# Autodesk Inventor assembly: Assembly1
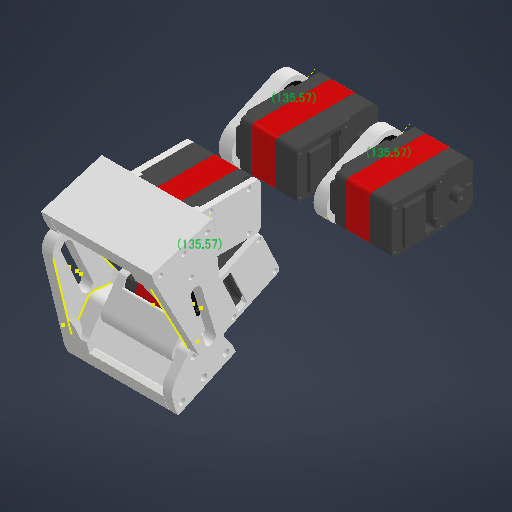
[picture p0: Inventor's stored thumbnail of the model, 512x512]
Saved by Autodesk Inventor 2026 (Build 300175000, 175)
## iProperties
Created: 2025-12-05
Part Number: Assembly1
Document SubType Name: Assembly
Designer: numai
Author: numai
## Documents named in this file (8)
- C:\Users\numai\Documents\workspace\inventor\feetech_slider_3dprint\Assembly1.iam
- C:\Users\numai\Documents\workspace\inventor\feetech_slider_3dprint\HLS3950M.ipt
- C:\Users\numai\Documents\workspace\inventor\feetech_slider_3dprint\ARRMA_1_7_25t_servo_arm.ipt
- C:\Users\numai\Documents\workspace\inventor\feetech_slider_3dprint\servo_side_plate1.ipt
- C:\Users\numai\Documents\workspace\inventor\feetech_slider_3dprint\servo_side_plate2.ipt
- C:\Users\numai\Documents\workspace\inventor\feetech_slider_3dprint\guideline.ipt
- C:\Users\numai\Documents\workspace\inventor\feetech_slider_3dprint\guideline_mir.ipt
- C:\Users\numai\Documents\workspace\inventor\feetech_slider_3dprint\arrma_boolean.ipt
## Components (17 placed, 7 different names)
1. HLS3950M:1 — メイト:1, メイト:2, フラッシュ:1, フラッシュ:2, フラッシュ:3, メイト:9, フラッシュ:4, フラッシュ:5
2. ARRMA_1_7_25t_servo_arm:1 — メイト:1, メイト:2, メイト:4
3. servo_side_plate1:1 — フラッシュ:1, フラッシュ:2
4. servo_side_plate2:1 — フラッシュ:3, メイト:23
5. guideline:1 — メイト:4, メイト:6, メイト:7, メイト:8
6. guideline_mir:1 — メイト:6, メイト:7, メイト:8, メイト:23
7. HLS3950M:2 — メイト:9, フラッシュ:4, フラッシュ:5, フラッシュ:6, フラッシュ:7, メイト:10, メイト:11, メイト:21, フラッシュ:8
8. HLS3950M:3 — フラッシュ:6, フラッシュ:7, メイト:12, メイト:13
9. ARRMA_1_7_25t_servo_arm:2 — メイト:10, メイト:11, メイト:14, メイト:18, メイト:19, メイト:20
10. ARRMA_1_7_25t_servo_arm:3 — メイト:12, メイト:13, メイト:14, メイト:15, メイト:16, メイト:17
11. arrma_boolean:1 — メイト:15, メイト:16, メイト:17, メイト:21
12. arrma_boolean:2 — メイト:18, メイト:19, メイト:20, メイト:24, フラッシュ:25
13. HLS3950M:4 — フラッシュ:8, メイト:24, フラッシュ:25, メイト:25, メイト:26, 角度:1, メイト:27, メイト:29
14. servo_side_plate1:2 — メイト:25, メイト:26, 角度:1, メイト:28, メイト:30, メイト:31
15. servo_side_plate2:2 — メイト:27, メイト:28, メイト:29
16. guideline:2 — メイト:30, メイト:31, メイト:32, メイト:33, メイト:34
17. guideline_mir:2 — メイト:32, メイト:33, メイト:34
## Relationships (41: Mate 31, Flush 9, Angle 1)
- メイト:1 [Mate]: HLS3950M:1 ↔ ARRMA_1_7_25t_servo_arm:1
- メイト:2 [Mate] (0.4 mm): HLS3950M:1 ↔ ARRMA_1_7_25t_servo_arm:1
- フラッシュ:1 [Flush]: HLS3950M:1 ↔ servo_side_plate1:1
- フラッシュ:2 [Flush]: HLS3950M:1 ↔ servo_side_plate1:1
- フラッシュ:3 [Flush]: HLS3950M:1 ↔ servo_side_plate2:1
- メイト:4 [Mate] (1 mm): ARRMA_1_7_25t_servo_arm:1 ↔ guideline:1
- メイト:6 [Mate]: guideline:1 ↔ guideline_mir:1
- メイト:7 [Mate]: guideline:1 ↔ guideline_mir:1
- メイト:8 [Mate]: guideline:1 ↔ guideline_mir:1
- メイト:9 [Mate] (22.48 mm): HLS3950M:1 ↔ HLS3950M:2
- フラッシュ:4 [Flush]: HLS3950M:1 ↔ HLS3950M:2
- フラッシュ:5 [Flush]: HLS3950M:1 ↔ HLS3950M:2
- フラッシュ:6 [Flush]: HLS3950M:2 ↔ HLS3950M:3
- フラッシュ:7 [Flush]: HLS3950M:2 ↔ HLS3950M:3
- メイト:10 [Mate] (0.4 mm): HLS3950M:2 ↔ ARRMA_1_7_25t_servo_arm:2
- メイト:11 [Mate]: HLS3950M:2 ↔ ARRMA_1_7_25t_servo_arm:2
- メイト:12 [Mate] (0.4 mm): HLS3950M:3 ↔ ARRMA_1_7_25t_servo_arm:3
- メイト:13 [Mate]: HLS3950M:3 ↔ ARRMA_1_7_25t_servo_arm:3
- メイト:14 [Mate]: ARRMA_1_7_25t_servo_arm:2 ↔ ARRMA_1_7_25t_servo_arm:3
- メイト:15 [Mate]: ARRMA_1_7_25t_servo_arm:3 ↔ arrma_boolean:1
- メイト:16 [Mate]: ARRMA_1_7_25t_servo_arm:3 ↔ arrma_boolean:1
- メイト:17 [Mate]: ARRMA_1_7_25t_servo_arm:3 ↔ arrma_boolean:1
- メイト:18 [Mate]: ARRMA_1_7_25t_servo_arm:2 ↔ arrma_boolean:2
- メイト:19 [Mate]: ARRMA_1_7_25t_servo_arm:2 ↔ arrma_boolean:2
- メイト:20 [Mate]: ARRMA_1_7_25t_servo_arm:2 ↔ arrma_boolean:2
- メイト:21 [Mate] (3.3 mm): HLS3950M:2 ↔ arrma_boolean:1
- メイト:23 [Mate]: servo_side_plate2:1 ↔ guideline_mir:1
- フラッシュ:8 [Flush]: HLS3950M:2 ↔ HLS3950M:4
- メイト:24 [Mate]: arrma_boolean:2 ↔ HLS3950M:4
- フラッシュ:25 [Flush] (80.2 mm): arrma_boolean:2 ↔ HLS3950M:4
- メイト:25 [Mate]: HLS3950M:4 ↔ servo_side_plate1:2
- メイト:26 [Mate]: HLS3950M:4 ↔ servo_side_plate1:2
- 角度:1 [Angle] (0 deg): HLS3950M:4 ↔ servo_side_plate1:2
- メイト:27 [Mate]: HLS3950M:4 ↔ servo_side_plate2:2
- メイト:28 [Mate]: servo_side_plate1:2 ↔ servo_side_plate2:2
- メイト:29 [Mate]: HLS3950M:4 ↔ servo_side_plate2:2
- メイト:30 [Mate]: servo_side_plate1:2 ↔ guideline:2
- メイト:31 [Mate]: servo_side_plate1:2 ↔ guideline:2
- メイト:32 [Mate]: guideline:2 ↔ guideline_mir:2
- メイト:33 [Mate]: guideline:2 ↔ guideline_mir:2
- メイト:34 [Mate]: guideline:2 ↔ guideline_mir:2
